# Autodesk Inventor assembly: ASY TKS 3520 FDS way 1
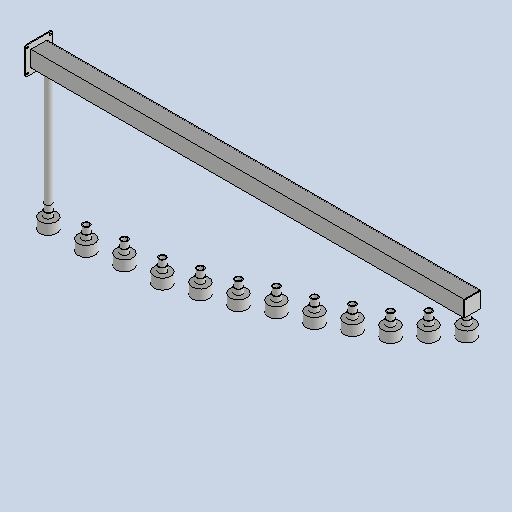
[picture p0: Inventor's stored thumbnail of the model, 512x512]
Saved by Autodesk Inventor 2025 (Build 290162010, 162A)
## iProperties
Created: 2025-07-02
Part Number: ASY TKS 3520 FDS way 1
Document SubType Name: Assembly
Designer: admin
Author: user
## Documents named in this file (7)
- C:\Users\admin\Yandex.Disk\home pc\Inventor\TKS-Tarko-Sale\BOTTOM DS\ASY TKS 3520 FDS way 1.iam
- C:\Users\admin\Yandex.Disk\home pc\Inventor\TKS-Tarko-Sale\BOTTOM DS\TKS 3521 FDS way 1.ipt
- C:\Users\admin\Yandex.Disk\home pc\Inventor\TKS-Tarko-Sale\BOTTOM DS\TKS dummy filter element.ipt
- C:\Users\admin\Yandex.Disk\home pc\Inventor\TKS-Tarko-Sale\BOTTOM DS\TKS dummy pipe nippel.ipt
- C:\Users\admin\Yandex.Disk\home pc\Inventor\TKS-Tarko-Sale\BOTTOM DS\TKS 3531 FDS Way FLANGE.ipt
- C:\Users\admin\Yandex.Disk\home pc\Inventor\TKS-Tarko-Sale\BOTTOM DS\TKS 3532 FDS way cup.ipt
- C:\Users\admin\Yandex.Disk\home pc\Inventor\TKS-Tarko-Sale\BOTTOM DS\TKS 3541 FDS thread  tube1.ipt
## Components (28 placed, 6 different names)
1. TKS 3521 FDS way 1.ipt:1 — Rigid:9, Rigid:10, Rotational:1, Rotational:2, Rotational:3, Rigid:21, Rigid:22, Rigid:23, Rigid:24, Rigid:25, Rigid:26, Rigid:27, Rigid:28, Rigid:29
2. TKS dummy filter element.ipt:1 — Rigid:1
3. TKS dummy pipe nippel.ipt:1 — Rigid:1, Rigid:22
4. TKS dummy filter element.ipt:2 — Rigid:3
5. TKS dummy pipe nippel.ipt:2 — Rigid:3, Rigid:29, Rigid:30
6. TKS dummy filter element.ipt:3 — Rigid:6
7. TKS dummy pipe nippel.ipt:3 — Rigid:6, Rotational:3
8. TKS 3531 FDS Way FLANGE.ipt:1 — Rigid:9
9. TKS 3532 FDS way cup.ipt:1 — Rigid:10
10. TKS dummy filter element.ipt:4 — Rigid:11
11. TKS dummy pipe nippel.ipt:4 — Rigid:11, Rigid:23
12. TKS dummy filter element.ipt:5 — Rigid:14
13. TKS dummy pipe nippel.ipt:5 — Rigid:14, Rotational:1
14. TKS dummy filter element.ipt:6
15. TKS dummy pipe nippel.ipt:6 — Rotational:2
16. TKS dummy filter element.ipt:7
17. TKS dummy pipe nippel.ipt:7 — Rigid:21
18. TKS dummy filter element.ipt:8
19. TKS dummy pipe nippel.ipt:8 — Rigid:28
20. TKS dummy filter element.ipt:9
21. TKS dummy pipe nippel.ipt:9 — Rigid:27
22. TKS dummy filter element.ipt:10
23. TKS dummy pipe nippel.ipt:10 — Rigid:26
24. TKS dummy filter element.ipt:11
25. TKS dummy pipe nippel.ipt:11 — Rigid:25
26. TKS dummy filter element.ipt:12
27. TKS dummy pipe nippel.ipt:12 — Rigid:24
28. TKS 3541 FDS thread  tube1.ipt:1 — Rigid:30
## Relationships (27: WeldJoint 24, RevoluteJoint 3)
- Rigid:1 [WeldJoint]: TKS dummy filter element.ipt:1 ↔ TKS dummy pipe nippel.ipt:1
- Rigid:3 [WeldJoint]: TKS dummy filter element.ipt:2 ↔ TKS dummy pipe nippel.ipt:2
- Rigid:6 [WeldJoint]: TKS dummy filter element.ipt:3 ↔ TKS dummy pipe nippel.ipt:3
- Rigid:9 [WeldJoint] (-3 mm): TKS 3521 FDS way 1.ipt:1 ↔ TKS 3531 FDS Way FLANGE.ipt:1
- Rigid:10 [WeldJoint]: TKS 3521 FDS way 1.ipt:1 ↔ TKS 3532 FDS way cup.ipt:1
- Rigid:11 [WeldJoint]: TKS dummy filter element.ipt:4 ↔ TKS dummy pipe nippel.ipt:4
- Rigid:14 [WeldJoint]: TKS dummy filter element.ipt:5 ↔ TKS dummy pipe nippel.ipt:5
- Rotational:1 [RevoluteJoint]: TKS 3521 FDS way 1.ipt:1 ↔ TKS dummy pipe nippel.ipt:5
- [WeldJoint]: TKS dummy filter element.ipt:6 ↔ TKS dummy pipe nippel.ipt:6
- [WeldJoint]: TKS dummy filter element.ipt:7 ↔ TKS dummy pipe nippel.ipt:7
- [WeldJoint]: TKS dummy filter element.ipt:8 ↔ TKS dummy pipe nippel.ipt:8
- [WeldJoint]: TKS dummy filter element.ipt:9 ↔ TKS dummy pipe nippel.ipt:9
- [WeldJoint]: TKS dummy filter element.ipt:10 ↔ TKS dummy pipe nippel.ipt:10
- [WeldJoint]: TKS dummy filter element.ipt:11 ↔ TKS dummy pipe nippel.ipt:11
- [WeldJoint]: TKS dummy filter element.ipt:12 ↔ TKS dummy pipe nippel.ipt:12
- Rotational:2 [RevoluteJoint] (-60 mm): TKS 3521 FDS way 1.ipt:1 ↔ TKS dummy pipe nippel.ipt:6
- Rotational:3 [RevoluteJoint] (-120 mm): TKS 3521 FDS way 1.ipt:1 ↔ TKS dummy pipe nippel.ipt:3
- Rigid:21 [WeldJoint] (-160 mm): TKS 3521 FDS way 1.ipt:1 ↔ TKS dummy pipe nippel.ipt:7
- Rigid:22 [WeldJoint] (-200 mm): TKS 3521 FDS way 1.ipt:1 ↔ TKS dummy pipe nippel.ipt:1
- Rigid:23 [WeldJoint] (-230 mm): TKS 3521 FDS way 1.ipt:1 ↔ TKS dummy pipe nippel.ipt:4
- Rigid:24 [WeldJoint] (-270 mm): TKS 3521 FDS way 1.ipt:1 ↔ TKS dummy pipe nippel.ipt:12
- Rigid:25 [WeldJoint] (-300 mm): TKS 3521 FDS way 1.ipt:1 ↔ TKS dummy pipe nippel.ipt:11
- Rigid:26 [WeldJoint] (-330 mm): TKS 3521 FDS way 1.ipt:1 ↔ TKS dummy pipe nippel.ipt:10
- Rigid:27 [WeldJoint] (-340 mm): TKS 3521 FDS way 1.ipt:1 ↔ TKS dummy pipe nippel.ipt:9
- Rigid:28 [WeldJoint] (-360 mm): TKS 3521 FDS way 1.ipt:1 ↔ TKS dummy pipe nippel.ipt:8
- Rigid:29 [WeldJoint] (-360 mm): TKS 3521 FDS way 1.ipt:1 ↔ TKS dummy pipe nippel.ipt:2
- Rigid:30 [WeldJoint]: TKS dummy pipe nippel.ipt:2 ↔ TKS 3541 FDS thread  tube1.ipt:1
## Named parameters: d19_d9 = 0 mm, d20_d9 = 0 mm, d21_d9 = 0 mm, d22_d9 = 0 mm, d23_d9 = 0 mm, d24_d9 = 0 mm, d25_d9 = 0 mm
